# Autodesk Inventor assembly: Nozzle
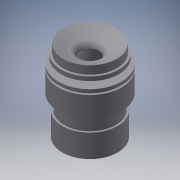
[picture p0: Inventor's stored thumbnail of the model, 180x180]
Saved by Autodesk Inventor 2017 (Build 210142000, 142)
## iProperties
Created: 2016-07-19
Part Number: Nozzle
Document SubType Name: Assembly
Designer: Bill
Author: Bill
## Documents named in this file (6)
- C:\Users\Bill\Desktop\NEW NEW\Nozzle.iam
- C:\Users\Bill\Desktop\NEW NEW\Carrier.ipt
- C:\Users\Bill\Desktop\NEW NEW\Graphite.ipt
- C:\Users\Bill\Desktop\NEW NEW\Phenlic.ipt
- C:\Users\Bill\Desktop\NEW NEW\Skirt.ipt
- C:\Users\Bill\Desktop\NEW NEW\Retainer.ipt
## Components (5 placed, 5 different names)
1. Carrier:1 — Mate:1, Mate:4, Mate:5, Mate:6, Mate:7
2. Graphite:1 — Mate:2, Mate:3
3. Phenlic:1 — Mate:1, Mate:2, Mate:3
4. Skirt:1 — Mate:4, Mate:5
5. Retainer:1 — Mate:6, Mate:7
## Relationships (7: Mate 7)
- Mate:1: Carrier:1 ↔ Phenlic:1
- Mate:2: Graphite:1 ↔ Phenlic:1
- Mate:3: Graphite:1 ↔ Phenlic:1
- Mate:4: Carrier:1 ↔ Skirt:1
- Mate:5: Carrier:1 ↔ Skirt:1
- Mate:6: Carrier:1 ↔ Retainer:1
- Mate:7: Carrier:1 ↔ Retainer:1
